# Autodesk Inventor assembly: Hexagonal Deco Lamp Assembly 175 thicker wall
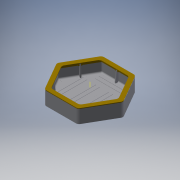
[picture p0: Inventor's stored thumbnail of the model, 180x180]
Saved by Autodesk Inventor 2019 (Build 230136000, 136)
## iProperties
Created: 2021-08-12
Part Number: Hexagonal Deco Lamp Assembly 175 thicker wall
Document SubType Name: Assembly
Designer: Lix
Author: Lix
## Documents named in this file (3)
- G:\Project\Hybrids\HexaWall\Inventor\Hexagonal Deco Lamp Assembly 175 thicker wall.iam
- G:\Project\Hybrids\HexaWall\Inventor\Base v6 - 175 - thicker wall.ipt
- G:\Project\Hybrids\HexaWall\Inventor\Cover v1 - 175 - 12mm rim - for thicker wall.ipt
## Components (2 placed, 2 different names)
1. Base v6 - 175 - thicker wall:1 — Mate:1, Mate:2, Mate:3
2. Cover v1 - 175 - 12mm rim - for thicker wall:1 — Mate:1, Mate:2, Mate:3
## Relationships (3: Mate 3)
- Mate:1: Base v6 - 175 - thicker wall:1 ↔ Cover v1 - 175 - 12mm rim - for thicker wall:1
- Mate:2: Base v6 - 175 - thicker wall:1 ↔ Cover v1 - 175 - 12mm rim - for thicker wall:1
- Mate:3: Base v6 - 175 - thicker wall:1 ↔ Cover v1 - 175 - 12mm rim - for thicker wall:1
